# Autodesk Inventor assembly: WheelAndTyre
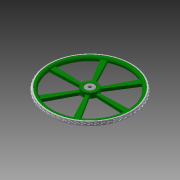
[picture p0: Inventor's stored thumbnail of the model, 180x180]
Saved by Autodesk Inventor 2014 SP1 (Build 180222100, 222)
## iProperties
Created: 2017-01-16
Part Number: WheelAndTyre
Document SubType Name: Assembly
Designer: danielsikar
Author: danielsikar
## Documents named in this file (4)
- C:\Users\danielsikar\Documents\Inventor\IoT-Trike\Assemblies\WheelTyre624Bearing.iam
- C:\Users\danielsikar\Documents\Inventor\IoT-Trike\Parts\WheelDia120.ipt
- C:\Users\danielsikar\Documents\Inventor\IoT-Trike\Parts\TyreR56mm.ipt
- C:\Users\danielsikar\Documents\Inventor\IoT-Trike\Parts\624Bearing.ipt
## Components (3 placed, 3 different names)
1. WheelDia120:1 — Mate:1, Mate:2, Mate:3, Flush:1, Mate:4, Flush:2
2. TyreR56mm:1 — Mate:3, Flush:1
3. 624Bearing:1 — Mate:4, Flush:2
## Relationships (6: Mate 4, Flush 2)
- Mate:1: WheelDia120:1
- Mate:2: WheelDia120:1
- Mate:3: WheelDia120:1 ↔ TyreR56mm:1
- Flush:1: WheelDia120:1 ↔ TyreR56mm:1
- Mate:4: WheelDia120:1 ↔ 624Bearing:1
- Flush:2: WheelDia120:1 ↔ 624Bearing:1
